# Autodesk Inventor assembly: Chassis-ver7-1111-2019
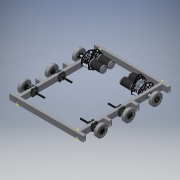
[picture p0: Inventor's stored thumbnail of the model, 180x180]
Saved by Autodesk Inventor 2018 (Build 220112000, 112)
## iProperties
Created: 2019-10-10
Part Number: Chassis-ver7-1111-2019
Document SubType Name: Assembly
Designer: JMHal
Author: JMHal
## Documents named in this file (9)
- E:\GrabCad\2019 - 2020 Off Season\TestChassis\Assembly\Chassis-ver7-1111-2019.iam
- E:\GrabCad\2019 - 2020 Off Season\TestChassis\Parts\2x1 20in Alluminum with Cal Drop.ver1-1111-2019.ipt
- E:\GrabCad\2019 - 2020 Off Season\TestChassis\Parts\2x1 20in Alluminum.ver1-1111-2019.ipt
- E:\GrabCad\2019 - 2020 Off Season\TestChassis\Parts\2x1 2in Alluminum Block.ver1-1111-2019.ipt
- E:\GrabCad\Resources\VEXpro Resources\Bearings\0.5inHexFlangedBearing(1.125inx0.313in)-1111-2016.ipt
- E:\GrabCad\Resources\VEXpro Resources\Versa Motion\VersaBlockKit-1111-2016.ipt
- E:\GrabCad\Resources\VEXpro Resources\Wheels\4 inch\4x1inTractionWheel(Tire)-1111-2016.iam
- E:\GrabCad\Resources\VEXpro Resources\Shafts\0.5inThunderHexShaft(8)-1111-2016.ipt
- E:\GrabCad\Resources\VEXpro Resources\Gearboxes\WCP SS Gearbox\SS-Gearbox.iam
## Components (40 placed, 8 different names)
1. 2x1 20in Alluminum with Cal Drop.ver1-1111-2019:1 — Mate:1, Mate:2, Mate:19, Mate:20, Mate:21, Mate:28, Mate:29, Mate:30, Mate:31, Mate:32, Mate:33, Mate:34, Mate:41, Mate:42, Insert:7, Mate:51, Insert:8, Angle:2, Mate:53, Angle:9, Insert:17, Angle:10, Insert:19, Angle:11, Mate:60, Cylindrical:1, Angle:16
2. 2x1 20in Alluminum.ver1-1111-2019:1 — Mate:1, Mate:2, Mate:3, Mate:5, Mate:6
3. 2x1 20in Alluminum with Cal Drop.ver1-1111-2019:2 — Mate:3, Mate:5, Mate:6, Mate:7, Mate:8, Mate:9, Mate:22, Mate:23, Mate:24, Mate:25, Mate:26, Mate:27, Mate:35, Mate:36, Mate:37, Mate:38, Mate:39, Mate:40, Insert:4, Insert:5, Angle:7, Angle:8, Insert:23, Angle:13, Insert:25, Angle:14, Rotational:1, Angle:17
4. 2x1 20in Alluminum.ver1-1111-2019:2 — Mate:7, Mate:8, Mate:9
5. 0.5inThunderHexShaft(8)-1111-2016:1 — Cylindrical:2, Rotational:9
6. SS-Gearbox:1 [sub-assembly] — Rotational:1, Angle:17, Rotational:2
7. SS-Gearbox:2 [sub-assembly] — Mate:60, Cylindrical:1, Angle:16, Cylindrical:11, Mate:61
8. 0.5inThunderHexShaft(8)-1111-2016:2 — Cylindrical:3, Rotational:8
9. 0.5inThunderHexShaft(8)-1111-2016:3 — Rotational:16, Rotational:4
10. 0.5inThunderHexShaft(8)-1111-2016:4 — Rotational:14, Rotational:13
11. 0.5inHexFlangedBearing(1.125inx0.313in)-1111-2016:20 — Rotational:14
12. 0.5inHexFlangedBearing(1.125inx0.313in)-1111-2016:19 — Rotational:16
13. 0.5inHexFlangedBearing(1.125inx0.313in)-1111-2016:6 — Insert:4, Mate:46, Mate:47
14. 0.5inHexFlangedBearing(1.125inx0.313in)-1111-2016:7 — Insert:5, Mate:48, Mate:49
15. 0.5inHexFlangedBearing(1.125inx0.313in)-1111-2016:17 — Insert:19, Cylindrical:3
16. 0.5inHexFlangedBearing(1.125inx0.313in)-1111-2016:16 — Insert:16, Insert:17, Cylindrical:2
17. 0.5inHexFlangedBearing(1.125inx0.313in)-1111-2016:9 — Insert:7, Mate:50, Mate:63
18. 0.5inHexFlangedBearing(1.125inx0.313in)-1111-2016:10 — Insert:8, Mate:52, Mate:62
19. 2x1 2in Alluminum Block.ver1-1111-2019:1 — Mate:22, Mate:23, Mate:24
20. 2x1 2in Alluminum Block.ver1-1111-2019:2 — Mate:19, Mate:20, Mate:21
21. 2x1 2in Alluminum Block.ver1-1111-2019:3 — Mate:25, Mate:26, Mate:27
22. 2x1 2in Alluminum Block.ver1-1111-2019:4 — Mate:28, Mate:29, Mate:30
23. 2x1 2in Alluminum Block.ver1-1111-2019:5 — Mate:31, Mate:32, Mate:41
24. 2x1 2in Alluminum Block.ver1-1111-2019:6 — Mate:33, Mate:34, Mate:42
25. 2x1 2in Alluminum Block.ver1-1111-2019:7 — Mate:35, Mate:36, Mate:40
26. 2x1 2in Alluminum Block.ver1-1111-2019:8 — Mate:37, Mate:38, Mate:39
27. VersaBlockKit-1111-2016:2 — Mate:46, Mate:47, Angle:8
28. VersaBlockKit-1111-2016:3 — Mate:48, Mate:49, Angle:7
29. VersaBlockKit-1111-2016:5 — Mate:50, Mate:51, Angle:2
30. VersaBlockKit-1111-2016:6 — Mate:52, Mate:53, Angle:9
31. VersaBlockKit-1111-2016:8 — Insert:16, Angle:10
32. VersaBlockKit-1111-2016:9 — Angle:11
33. VersaBlockKit-1111-2016:11 — Insert:23, Angle:13
34. VersaBlockKit-1111-2016:12 — Insert:25, Angle:14
35. 4x1inTractionWheel(Tire)-1111-2016:1 [sub-assembly] — Rotational:2
36. 4x1inTractionWheel(Tire)-1111-2016:2 [sub-assembly] — Rotational:13
37. 4x1inTractionWheel(Tire)-1111-2016:3 [sub-assembly] — Rotational:4
38. 4x1inTractionWheel(Tire)-1111-2016:4 [sub-assembly] — Cylindrical:11, Mate:61
39. 4x1inTractionWheel(Tire)-1111-2016:5 [sub-assembly] — Rotational:9, Mate:63
40. 4x1inTractionWheel(Tire)-1111-2016:6 [sub-assembly] — Rotational:8, Mate:62
## Relationships (82: Mate 48, Insert 12, Angle 10, RevoluteJoint 8, CylindricalJoint 4)
- Mate:1: 2x1 20in Alluminum with Cal Drop.ver1-1111-2019:1 ↔ 2x1 20in Alluminum.ver1-1111-2019:1
- Mate:2: 2x1 20in Alluminum with Cal Drop.ver1-1111-2019:1 ↔ 2x1 20in Alluminum.ver1-1111-2019:1
- Mate:3: 2x1 20in Alluminum.ver1-1111-2019:1 ↔ 2x1 20in Alluminum with Cal Drop.ver1-1111-2019:2
- Mate:5: 2x1 20in Alluminum.ver1-1111-2019:1 ↔ 2x1 20in Alluminum with Cal Drop.ver1-1111-2019:2
- Mate:6: 2x1 20in Alluminum.ver1-1111-2019:1 ↔ 2x1 20in Alluminum with Cal Drop.ver1-1111-2019:2
- Mate:7: 2x1 20in Alluminum with Cal Drop.ver1-1111-2019:2 ↔ 2x1 20in Alluminum.ver1-1111-2019:2
- Mate:8: 2x1 20in Alluminum with Cal Drop.ver1-1111-2019:2 ↔ 2x1 20in Alluminum.ver1-1111-2019:2
- Mate:9: 2x1 20in Alluminum with Cal Drop.ver1-1111-2019:2 ↔ 2x1 20in Alluminum.ver1-1111-2019:2
- Mate:19: 2x1 20in Alluminum with Cal Drop.ver1-1111-2019:1 ↔ 2x1 2in Alluminum Block.ver1-1111-2019:2
- Mate:20: 2x1 20in Alluminum with Cal Drop.ver1-1111-2019:1 ↔ 2x1 2in Alluminum Block.ver1-1111-2019:2
- Mate:21: 2x1 20in Alluminum with Cal Drop.ver1-1111-2019:1 ↔ 2x1 2in Alluminum Block.ver1-1111-2019:2
- Mate:22: 2x1 20in Alluminum with Cal Drop.ver1-1111-2019:2 ↔ 2x1 2in Alluminum Block.ver1-1111-2019:1
- Mate:23: 2x1 20in Alluminum with Cal Drop.ver1-1111-2019:2 ↔ 2x1 2in Alluminum Block.ver1-1111-2019:1
- Mate:24: 2x1 20in Alluminum with Cal Drop.ver1-1111-2019:2 ↔ 2x1 2in Alluminum Block.ver1-1111-2019:1
- Mate:25: 2x1 20in Alluminum with Cal Drop.ver1-1111-2019:2 ↔ 2x1 2in Alluminum Block.ver1-1111-2019:3
- Mate:26: 2x1 20in Alluminum with Cal Drop.ver1-1111-2019:2 ↔ 2x1 2in Alluminum Block.ver1-1111-2019:3
- Mate:27: 2x1 20in Alluminum with Cal Drop.ver1-1111-2019:2 ↔ 2x1 2in Alluminum Block.ver1-1111-2019:3
- Mate:28: 2x1 20in Alluminum with Cal Drop.ver1-1111-2019:1 ↔ 2x1 2in Alluminum Block.ver1-1111-2019:4
- Mate:29: 2x1 20in Alluminum with Cal Drop.ver1-1111-2019:1 ↔ 2x1 2in Alluminum Block.ver1-1111-2019:4
- Mate:30: 2x1 20in Alluminum with Cal Drop.ver1-1111-2019:1 ↔ 2x1 2in Alluminum Block.ver1-1111-2019:4
- Mate:31: 2x1 20in Alluminum with Cal Drop.ver1-1111-2019:1 ↔ 2x1 2in Alluminum Block.ver1-1111-2019:5
- Mate:32: 2x1 20in Alluminum with Cal Drop.ver1-1111-2019:1 ↔ 2x1 2in Alluminum Block.ver1-1111-2019:5
- Mate:33: 2x1 20in Alluminum with Cal Drop.ver1-1111-2019:1 ↔ 2x1 2in Alluminum Block.ver1-1111-2019:6
- Mate:34: 2x1 20in Alluminum with Cal Drop.ver1-1111-2019:1 ↔ 2x1 2in Alluminum Block.ver1-1111-2019:6
- Mate:35: 2x1 20in Alluminum with Cal Drop.ver1-1111-2019:2 ↔ 2x1 2in Alluminum Block.ver1-1111-2019:7
- Mate:36: 2x1 20in Alluminum with Cal Drop.ver1-1111-2019:2 ↔ 2x1 2in Alluminum Block.ver1-1111-2019:7
- Mate:37: 2x1 20in Alluminum with Cal Drop.ver1-1111-2019:2 ↔ 2x1 2in Alluminum Block.ver1-1111-2019:8
- Mate:38: 2x1 20in Alluminum with Cal Drop.ver1-1111-2019:2 ↔ 2x1 2in Alluminum Block.ver1-1111-2019:8
- Mate:39 (139.7 mm): 2x1 20in Alluminum with Cal Drop.ver1-1111-2019:2 ↔ 2x1 2in Alluminum Block.ver1-1111-2019:8
- Mate:40 (139.7 mm): 2x1 20in Alluminum with Cal Drop.ver1-1111-2019:2 ↔ 2x1 2in Alluminum Block.ver1-1111-2019:7
- Mate:41 (139.7 mm): 2x1 20in Alluminum with Cal Drop.ver1-1111-2019:1 ↔ 2x1 2in Alluminum Block.ver1-1111-2019:5
- Mate:42 (139.7 mm): 2x1 20in Alluminum with Cal Drop.ver1-1111-2019:1 ↔ 2x1 2in Alluminum Block.ver1-1111-2019:6
- Insert:4: 2x1 20in Alluminum with Cal Drop.ver1-1111-2019:2 ↔ 0.5inHexFlangedBearing(1.125inx0.313in)-1111-2016:6
- Mate:46: 0.5inHexFlangedBearing(1.125inx0.313in)-1111-2016:6 ↔ VersaBlockKit-1111-2016:2
- Mate:47: 0.5inHexFlangedBearing(1.125inx0.313in)-1111-2016:6 ↔ VersaBlockKit-1111-2016:2
- Insert:5: 2x1 20in Alluminum with Cal Drop.ver1-1111-2019:2 ↔ 0.5inHexFlangedBearing(1.125inx0.313in)-1111-2016:7
- Mate:48: 0.5inHexFlangedBearing(1.125inx0.313in)-1111-2016:7 ↔ VersaBlockKit-1111-2016:3
- Mate:49: 0.5inHexFlangedBearing(1.125inx0.313in)-1111-2016:7 ↔ VersaBlockKit-1111-2016:3
- Insert:7: 2x1 20in Alluminum with Cal Drop.ver1-1111-2019:1 ↔ 0.5inHexFlangedBearing(1.125inx0.313in)-1111-2016:9
- Mate:50: 0.5inHexFlangedBearing(1.125inx0.313in)-1111-2016:9 ↔ VersaBlockKit-1111-2016:5
- Mate:51: 2x1 20in Alluminum with Cal Drop.ver1-1111-2019:1 ↔ VersaBlockKit-1111-2016:5
- Insert:8: 2x1 20in Alluminum with Cal Drop.ver1-1111-2019:1 ↔ 0.5inHexFlangedBearing(1.125inx0.313in)-1111-2016:10
- Angle:2 (0 deg): 2x1 20in Alluminum with Cal Drop.ver1-1111-2019:1 ↔ VersaBlockKit-1111-2016:5
- Angle:7 (0 deg): 2x1 20in Alluminum with Cal Drop.ver1-1111-2019:2 ↔ VersaBlockKit-1111-2016:3
- Angle:8 (0 deg): 2x1 20in Alluminum with Cal Drop.ver1-1111-2019:2 ↔ VersaBlockKit-1111-2016:2
- Mate:52: 0.5inHexFlangedBearing(1.125inx0.313in)-1111-2016:10 ↔ VersaBlockKit-1111-2016:6
- Mate:53: 2x1 20in Alluminum with Cal Drop.ver1-1111-2019:1 ↔ VersaBlockKit-1111-2016:6
- Angle:9 (0 deg): 2x1 20in Alluminum with Cal Drop.ver1-1111-2019:1 ↔ VersaBlockKit-1111-2016:6
- [Mate]: 0.5inHexFlangedBearing(1.125inx0.313in)-1111-2016:16 ↔ VersaBlockKit-1111-2016:8
- Insert:16: 0.5inHexFlangedBearing(1.125inx0.313in)-1111-2016:16 ↔ VersaBlockKit-1111-2016:8
- Insert:17: 2x1 20in Alluminum with Cal Drop.ver1-1111-2019:1 ↔ 0.5inHexFlangedBearing(1.125inx0.313in)-1111-2016:16
- Angle:10 (0 deg): 2x1 20in Alluminum with Cal Drop.ver1-1111-2019:1 ↔ VersaBlockKit-1111-2016:8
- [Mate]: 0.5inHexFlangedBearing(1.125inx0.313in)-1111-2016:17 ↔ VersaBlockKit-1111-2016:9
- [Insert]: 0.5inHexFlangedBearing(1.125inx0.313in)-1111-2016:17 ↔ VersaBlockKit-1111-2016:9
- Insert:19: 2x1 20in Alluminum with Cal Drop.ver1-1111-2019:1 ↔ 0.5inHexFlangedBearing(1.125inx0.313in)-1111-2016:17
- Angle:11 (0 deg): 2x1 20in Alluminum with Cal Drop.ver1-1111-2019:1 ↔ VersaBlockKit-1111-2016:9
- [Mate]: 0.5inHexFlangedBearing(1.125inx0.313in)-1111-2016:19 ↔ VersaBlockKit-1111-2016:11
- [Insert]: 0.5inHexFlangedBearing(1.125inx0.313in)-1111-2016:19 ↔ VersaBlockKit-1111-2016:11
- Insert:23: 2x1 20in Alluminum with Cal Drop.ver1-1111-2019:2 ↔ VersaBlockKit-1111-2016:11
- Angle:13 (0 deg): 2x1 20in Alluminum with Cal Drop.ver1-1111-2019:2 ↔ VersaBlockKit-1111-2016:11
- [Mate]: 0.5inHexFlangedBearing(1.125inx0.313in)-1111-2016:20 ↔ VersaBlockKit-1111-2016:12
- [Insert]: 0.5inHexFlangedBearing(1.125inx0.313in)-1111-2016:20 ↔ VersaBlockKit-1111-2016:12
- Insert:25: 2x1 20in Alluminum with Cal Drop.ver1-1111-2019:2 ↔ VersaBlockKit-1111-2016:12
- Angle:14 (0 deg): 2x1 20in Alluminum with Cal Drop.ver1-1111-2019:2 ↔ VersaBlockKit-1111-2016:12
- Mate:60: 2x1 20in Alluminum with Cal Drop.ver1-1111-2019:1 ↔ SS-Gearbox:2
- Cylindrical:1: 2x1 20in Alluminum with Cal Drop.ver1-1111-2019:1 ↔ SS-Gearbox:2
- Cylindrical:2: 0.5inThunderHexShaft(8)-1111-2016:1 ↔ 0.5inHexFlangedBearing(1.125inx0.313in)-1111-2016:16
- Cylindrical:3: 0.5inThunderHexShaft(8)-1111-2016:2 ↔ 0.5inHexFlangedBearing(1.125inx0.313in)-1111-2016:17
- Rotational:16 [RevoluteJoint] (91.44 mm): 0.5inThunderHexShaft(8)-1111-2016:3 ↔ 0.5inHexFlangedBearing(1.125inx0.313in)-1111-2016:19
- Rotational:14 [RevoluteJoint] (91.44 mm): 0.5inThunderHexShaft(8)-1111-2016:4 ↔ 0.5inHexFlangedBearing(1.125inx0.313in)-1111-2016:20
- Angle:16 (90 deg): 2x1 20in Alluminum with Cal Drop.ver1-1111-2019:1 ↔ SS-Gearbox:2
- Rotational:1 [RevoluteJoint]: 2x1 20in Alluminum with Cal Drop.ver1-1111-2019:2 ↔ SS-Gearbox:1
- Angle:17 (90 deg): 2x1 20in Alluminum with Cal Drop.ver1-1111-2019:2 ↔ SS-Gearbox:1
- Rotational:2 [RevoluteJoint]: SS-Gearbox:1 ↔ 4x1inTractionWheel(Tire)-1111-2016:1
- Rotational:4 [RevoluteJoint]: 0.5inThunderHexShaft(8)-1111-2016:3 ↔ 4x1inTractionWheel(Tire)-1111-2016:3
- Cylindrical:11: SS-Gearbox:2 ↔ 4x1inTractionWheel(Tire)-1111-2016:4
- Rotational:9 [RevoluteJoint]: 0.5inThunderHexShaft(8)-1111-2016:1 ↔ 4x1inTractionWheel(Tire)-1111-2016:5
- Mate:61 (-74.93 mm): SS-Gearbox:2 ↔ 4x1inTractionWheel(Tire)-1111-2016:4
- Rotational:8 [RevoluteJoint]: 0.5inThunderHexShaft(8)-1111-2016:2 ↔ 4x1inTractionWheel(Tire)-1111-2016:6
- Mate:62 (-71.12 mm): 0.5inHexFlangedBearing(1.125inx0.313in)-1111-2016:10 ↔ 4x1inTractionWheel(Tire)-1111-2016:6
- Mate:63 (-74.422 mm): 0.5inHexFlangedBearing(1.125inx0.313in)-1111-2016:9 ↔ 4x1inTractionWheel(Tire)-1111-2016:5
- Rotational:13 [RevoluteJoint]: 0.5inThunderHexShaft(8)-1111-2016:4 ↔ 4x1inTractionWheel(Tire)-1111-2016:2
## Named parameters: d89_d76 = 0 mm, d93_d89_d76 = 0 mm, d94_d90 = 0 mm, d103_d89_d76 = 0 mm, d104_d90 = 0 mm, d107_d89_d76 = 0 mm, d108_d90 = 0 mm
